# Autodesk Inventor assembly: robot
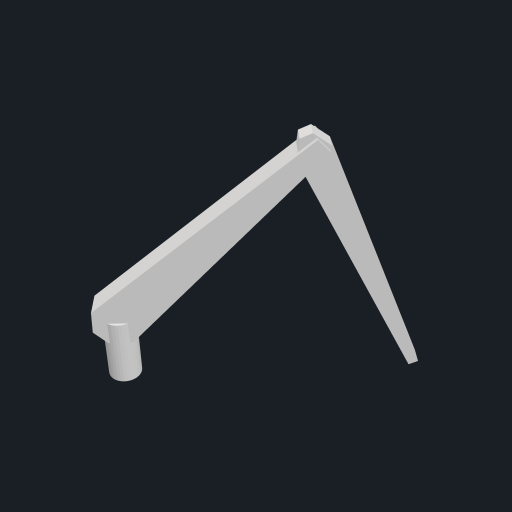
[picture p0: Inventor's stored thumbnail of the model, 512x512]
Saved by Autodesk Inventor 2023 (Build 270158000, 158)
## iProperties
Created: 2024-01-08
Part Number: robot
Document SubType Name: Assembly
Designer: valer
Mass: 3.06569e+06 g
Surface Area: 129954 cm^2
Volume: 1.13544e+06 cm^3
Density: 2.7 g/cm^3
Author: valer
## Documents named in this file (4)
- C:\Users\valer\Desktop\basic_velocity_control\description\cad\robot.iam
- C:\Users\valer\Desktop\basic_velocity_control\description\cad\shoulder.ipt
- C:\Users\valer\Desktop\basic_velocity_control\description\cad\upperarm.ipt
- C:\Users\valer\Desktop\basic_velocity_control\description\cad\forearm.ipt
## Components (3 placed, 3 different names)
1. shoulder:1 — Mate:1, Mate:2, Mate:4, Mate:5
2. upperarm:1 — Mate:4, Mate:5, Mate:6, Mate:7
3. forearm:1 — Mate:6, Mate:7
## Relationships (6: Mate 6)
- Mate:1: shoulder:1
- Mate:2: shoulder:1
- Mate:4: shoulder:1 ↔ upperarm:1
- Mate:5: shoulder:1 ↔ upperarm:1
- Mate:6: upperarm:1 ↔ forearm:1
- Mate:7: upperarm:1 ↔ forearm:1
